# Autodesk Inventor assembly: Tweepr
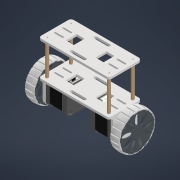
[picture p0: Inventor's stored thumbnail of the model, 180x180]
Saved by Autodesk Inventor 2022.1 (Build 261234000, 234)
## iProperties
Created: 2021-10-11
Part Number: Tweepr
Document SubType Name: Assembly
Designer: Santiago Martínez
Mass: 264.628 g
Surface Area: 1447.95 cm^2
Volume: 240.891 cm^3
Density: 1.09854 g/cm^3
Author: Santiago Martínez
## Documents named in this file (7)
- D:\Santiago\Documents\My Works\Universidad de Los Andes\Proyecto de Grado IELE\3- CAD\Tweepr.iam
- D:\Santiago\Documents\My Works\Universidad de Los Andes\Proyecto de Grado IELE\3- CAD\Base.ipt
- D:\Santiago\Documents\My Works\Universidad de Los Andes\Proyecto de Grado IELE\3- CAD\Standart Parts\Nema 17 Stepper (17HS4401)17HS4401 Nema 17 Stepper.iam
- D:\Santiago\Documents\My Works\Universidad de Los Andes\Proyecto de Grado IELE\3- CAD\Brass Spacer.ipt
- D:\Santiago\Documents\My Works\Universidad de Los Andes\Proyecto de Grado IELE\3- CAD\Top.ipt
- D:\Santiago\Documents\My Works\Universidad de Los Andes\Proyecto de Grado IELE\3- CAD\Wheel Outer.ipt
- D:\Santiago\Documents\My Works\Universidad de Los Andes\Proyecto de Grado IELE\3- CAD\Wheel Inside.ipt
## Components (12 placed, 6 different names)
1. Base:1 — Mate:1, Mate:2, Mate:3, Mate:4, Mate:5, Mate:6, Mate:7, Mate:8, Mate:9, Mate:10, Mate:11, Mate:12, Mate:13, Mate:14, Mate:15, Mate:16, Angle:1, Angle:2, Angle:3, Angle:4, Angle:5, Angle:6
2. Nema 17 Stepper (17HS4401)17HS4401 Nema 17 Stepper:1 [sub-assembly] — Mate:5, Mate:6, Mate:7, Mate:8, Mate:22, Mate:23
3. Nema 17 Stepper (17HS4401)17HS4401 Nema 17 Stepper:2 [sub-assembly] — Mate:1, Mate:2, Mate:3, Mate:4, Mate:24, Mate:25
4. Brass Spacer:1 — Mate:11, Mate:16, Angle:2, Mate:20
5. Brass Spacer:2 — Mate:12, Mate:13, Angle:1, Mate:19
6. Brass Spacer:3 — Mate:9, Mate:15, Angle:3, Mate:17, Mate:21
7. Brass Spacer:4 — Mate:10, Mate:14, Angle:4, Mate:18
8. Top:1 — Mate:17, Mate:18, Mate:19, Mate:20, Mate:21
9. Wheel Inside:1 — Mate:22, Mate:23, Angle:6, Mate:26, Flush:1
10. Wheel Inside:2 — Mate:24, Mate:25, Angle:5, Mate:27, Flush:2
11. Wheel Outer:1 — Mate:27, Flush:2
12. Wheel Outer:2 — Mate:26, Flush:1
## Relationships (35: Mate 27, Angle 6, Flush 2)
- Mate:1: Base:1 ↔ Nema 17 Stepper (17HS4401)17HS4401 Nema 17 Stepper:2
- Mate:2: Base:1 ↔ Nema 17 Stepper (17HS4401)17HS4401 Nema 17 Stepper:2
- Mate:3: Base:1 ↔ Nema 17 Stepper (17HS4401)17HS4401 Nema 17 Stepper:2
- Mate:4: Base:1 ↔ Nema 17 Stepper (17HS4401)17HS4401 Nema 17 Stepper:2
- Mate:5: Base:1 ↔ Nema 17 Stepper (17HS4401)17HS4401 Nema 17 Stepper:1
- Mate:6: Base:1 ↔ Nema 17 Stepper (17HS4401)17HS4401 Nema 17 Stepper:1
- Mate:7: Base:1 ↔ Nema 17 Stepper (17HS4401)17HS4401 Nema 17 Stepper:1
- Mate:8: Base:1 ↔ Nema 17 Stepper (17HS4401)17HS4401 Nema 17 Stepper:1
- Mate:9: Base:1 ↔ Brass Spacer:3
- Mate:10: Base:1 ↔ Brass Spacer:4
- Mate:11: Base:1 ↔ Brass Spacer:1
- Mate:12: Base:1 ↔ Brass Spacer:2
- Mate:13: Base:1 ↔ Brass Spacer:2
- Mate:14: Base:1 ↔ Brass Spacer:4
- Mate:15: Base:1 ↔ Brass Spacer:3
- Mate:16: Base:1 ↔ Brass Spacer:1
- Angle:1 (0 deg): Base:1 ↔ Brass Spacer:2
- Angle:2 (0 deg): Base:1 ↔ Brass Spacer:1
- Angle:3 (0 deg): Base:1 ↔ Brass Spacer:3
- Angle:4 (0 deg): Base:1 ↔ Brass Spacer:4
- Mate:17: Brass Spacer:3 ↔ Top:1
- Mate:18: Brass Spacer:4 ↔ Top:1
- Mate:19: Brass Spacer:2 ↔ Top:1
- Mate:20: Brass Spacer:1 ↔ Top:1
- Mate:21: Brass Spacer:3 ↔ Top:1
- Mate:22: Nema 17 Stepper (17HS4401)17HS4401 Nema 17 Stepper:1 ↔ Wheel Inside:1
- Mate:23: Nema 17 Stepper (17HS4401)17HS4401 Nema 17 Stepper:1 ↔ Wheel Inside:1
- Mate:24: Nema 17 Stepper (17HS4401)17HS4401 Nema 17 Stepper:2 ↔ Wheel Inside:2
- Mate:25: Nema 17 Stepper (17HS4401)17HS4401 Nema 17 Stepper:2 ↔ Wheel Inside:2
- Angle:5 (0 deg): Base:1 ↔ Wheel Inside:2
- Angle:6 (0 deg): Base:1 ↔ Wheel Inside:1
- Mate:26: Wheel Inside:1 ↔ Wheel Outer:2
- Flush:1: Wheel Inside:1 ↔ Wheel Outer:2
- Mate:27: Wheel Inside:2 ↔ Wheel Outer:1
- Flush:2: Wheel Inside:2 ↔ Wheel Outer:1
